# Autodesk Inventor assembly: servo
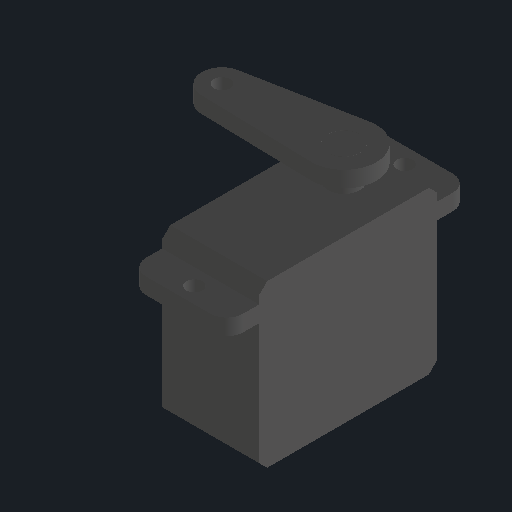
[picture p0: Inventor's stored thumbnail of the model, 512x512]
Saved by Autodesk Inventor 2023 (Build 270158030, 158C)
## iProperties
Created: 2022-03-30
Part Number: servo
Document SubType Name: Assembly
Designer: kardo
Author: kardo
## Documents named in this file (3)
- D:\Computer Aided Design\hydroplane_plan_2_refactor\model\shape\frame\hardware\servo.iam
- D:\Computer Aided Design\hydroplane_plan_2_refactor\model\shape\frame\hardware\servo_arm.ipt
- D:\Computer Aided Design\hydroplane_plan_2_refactor\model\shape\frame\hardware\servo_body.ipt
## Components (2 placed, 2 different names)
1. servo_arm:1 — Cylindrical:1
2. servo_body:1 — Cylindrical:1
## Relationships (1: CylindricalJoint 1)
- Cylindrical:1: servo_arm:1 ↔ servo_body:1
